# Autodesk Inventor assembly: V_Bearing
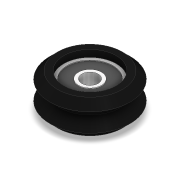
[picture p0: Inventor's stored thumbnail of the model, 180x180]
Saved by Autodesk Inventor 2020 (Build 240168000, 168)
## iProperties
Created: 2020-03-27
Part Number: V_Bearing
Document SubType Name: Assembly
Designer: chitl
Author: chitl
## Documents named in this file (3)
- C:\Users\chitl\Desktop\CNC-Drawing-Robot\Inventor Files\Y-Axis\V_Bearing.iam
- C:\Users\chitl\Desktop\CNC-Drawing-Robot\Inventor Files\Y-Axis\Ball Bearing 625 2RS 5x16x5.ipt
- C:\Users\chitl\Desktop\CNC-Drawing-Robot\Inventor Files\Y-Axis\Delrin V-Wheel.ipt
## Components (2 placed, 2 different names)
1. Ball Bearing 625 2RS 5x16x5:1 — Mate:1, Mate:2
2. Delrin V-Wheel:1 — Mate:1, Mate:2
## Relationships (2: Mate 2)
- Mate:1: Ball Bearing 625 2RS 5x16x5:1 ↔ Delrin V-Wheel:1
- Mate:2: Ball Bearing 625 2RS 5x16x5:1 ↔ Delrin V-Wheel:1
